# Autodesk Inventor assembly: new vial holder assembly
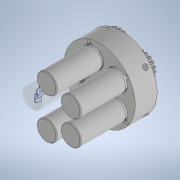
[picture p0: Inventor's stored thumbnail of the model, 180x180]
Saved by Autodesk Inventor 2022 (Build 260153000, 153)
## iProperties
Created: 2022-06-21
Part Number: new vial holder assembly
Document SubType Name: Assembly
Designer: efred
Author: efred
## Documents named in this file (8)
- C:\Users\efred\OneDrive - Imperial College London\ROBOICP\new vial holder assembly.iam
- C:\Users\efred\OneDrive - Imperial College London\ROBOICP\Final Assembly\vial.ipt
- C:\Users\efred\OneDrive - Imperial College London\ROBOICP\Old Files\roboICP-main\Reaction System\Vial assembly\vial thread insert.ipt
- C:\Users\efred\OneDrive - Imperial College London\ROBOICP\Final Assembly\STL Files\Vial upper holder.ipt
- C:\Users\efred\OneDrive - Imperial College London\ROBOICP\mixer_gear.ipt
- C:\Users\efred\OneDrive - Imperial College London\ROBOICP\Mixer.ipt
- C:\Users\efred\OneDrive - Imperial College London\ROBOICP\center_gear.ipt
- C:\Users\efred\OneDrive - Imperial College London\ROBOICP\Stirring motor.ipt
## Components (23 placed, 7 different names)
1. Vial upper holder:1 — Flush:2, Flush:3, Mate:3, Mate:5, Mate:6
2. center_gear:1 — Mate:5, Mate:6, Flush:7, Mate:7
3. Stirring motor:1 — Flush:7, Mate:7
4. vial thread insert:1 — Flush:1, Mate:1
5. vial:1 — Flush:1, Mate:1, Flush:2, Flush:3, Mate:2
6. mixer_gear:1 — Flush:5, Mate:2, Mate:3, Flush:6, Mate:4, Angle:1
7. Mixer:1 — Flush:6, Mate:4, Angle:1
8. vial thread insert:2
9. vial:2
10. mixer_gear:2
11. Mixer:2
12. vial thread insert:3
13. vial:3
14. mixer_gear:3
15. Mixer:3
16. vial thread insert:4
17. vial:4
18. mixer_gear:4
19. Mixer:4
20. vial thread insert:5
21. vial:5
22. mixer_gear:5
23. Mixer:5
## Component patterns: (5 elements, first: vial thread insert:1 + vial:1 + mixer_gear:1 + Mixer:1)
## Relationships (14: Mate 7, Flush 6, Angle 1)
- Flush:1 (-1 mm): vial thread insert:1 ↔ vial:1
- Mate:1: vial thread insert:1 ↔ vial:1
- Flush:2: Vial upper holder:1 ↔ vial:1
- Flush:3: Vial upper holder:1 ↔ vial:1
- Flush:5: mixer_gear:1
- Mate:2: vial:1 ↔ mixer_gear:1
- Mate:3 (0.1 mm): Vial upper holder:1 ↔ mixer_gear:1
- Flush:6: mixer_gear:1 ↔ Mixer:1
- Mate:4: mixer_gear:1 ↔ Mixer:1
- Angle:1 (0 deg): mixer_gear:1 ↔ Mixer:1
- Mate:5 (0.1 mm): Vial upper holder:1 ↔ center_gear:1
- Mate:6: Vial upper holder:1 ↔ center_gear:1
- Flush:7: center_gear:1 ↔ Stirring motor:1
- Mate:7: center_gear:1 ↔ Stirring motor:1
